# Autodesk Inventor assembly: RotaryBase
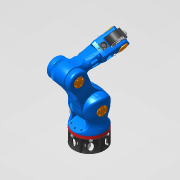
[picture p0: Inventor's stored thumbnail of the model, 180x180]
Saved by Autodesk Inventor 2014 SP2 (Build 180246200, 246)
## iProperties
Created: 2014-12-13
Part Number: RotaryBase
Document SubType Name: Assembly
Designer: 4ndreas
Author: 4ndreas
## Documents named in this file (12)
- C:\Users\4ndreas\Documents\Inventor\RobotARm\RotaryBase.iam
- C:\Users\4ndreas\Documents\Inventor\RobotARm\RotaryBase_B.ipt
- C:\Users\4ndreas\Documents\Inventor\Content Center Files\R2014\de-DE\DIN BEARING(1)\DIN 625 SKF - SKF 608.ipt
- C:\Users\4ndreas\Documents\Inventor\Content Center Files\R2014\de-DE\DIN 931-1\DIN 931-1 - M8 x 60.ipt
- C:\Users\4ndreas\Documents\Inventor\RobotARm\RotaryBase.ipt
- C:\Users\4ndreas\Documents\Inventor\Content Center Files\R2014\de-DE\DIN BEARING(1)\DIN 625 SKF - SKF 625.ipt
- C:\Users\4ndreas\Documents\Inventor\Content Center Files\R2014\de-DE\DIN 931-1\DIN 931-1 - M5 x 25.ipt
- C:\Users\4ndreas\Documents\Inventor\Content Center Files\R2014\de-DE\DIN 985\DIN 985 - M5.ipt
- C:\Users\4ndreas\Documents\Inventor\Content Center Files\R2014\de-DE\DIN 985\DIN 985 - M8.ipt
- C:\Users\4ndreas\Documents\Inventor\RobotARm\Nema17.ipt
- C:\Users\4ndreas\Documents\Inventor\RobotARm\MovingArm.iam
- C:\Users\4ndreas\Documents\Inventor\RobotARm\Stirnzahnrad_C_print.ipt
## Components (27 placed, 11 different names)
1. RotaryBase_B:1 — Fluchtend:1, Passend:1, Passend:2, Passend:3, Passend:4, Passend:5, Passend:6, Passend:8, Passend:9, Passend:13, Passend:16, Passend:17, Passend:18
2. DIN 625 SKF 608:1 — Passend:2, Passend:5
3. DIN 625 SKF 608:2 — Passend:3, Passend:4, Passend:15
4. DIN 931-1 - ersetzt durch DIN EN 24014 M8 x 60:1 — Passend:6, Passend:7, Fluchtend:2, Winkel:1, Passend:14
5. RotaryBase:1 — Passend:7, Tangential:1, Fluchtend:2, Winkel:1, Passend:19, Passend:20, Passend:21
6. DIN 985 - ersetzt durch DIN EN ISO 10511 M8:1 — Passend:14, Passend:15
7. Nema17:1 — Passend:16, Passend:17, Passend:18, Passend:22, Fluchtend:3
8. MovingArm:1 [sub-assembly] — Passend:19, Passend:20, Passend:21
9. Stirnzahnrad_C_print:1 — Passend:22, Fluchtend:3
10. DIN 625 SKF 625:1 — Passend:8, Passend:9, Tangential:1, Passend:10, Passend:11
11. DIN 931-1 - ersetzt durch DIN EN 24014 M5 x 25:1 — Passend:10, Passend:11, Passend:12
12. DIN 985 - ersetzt durch DIN EN ISO 10511 M5:1 — Passend:12, Passend:13
13. DIN 625 SKF 625:2
14. DIN 931-1 - ersetzt durch DIN EN 24014 M5 x 25:2
15. DIN 985 - ersetzt durch DIN EN ISO 10511 M5:2
16. DIN 625 SKF 625:3
17. DIN 931-1 - ersetzt durch DIN EN 24014 M5 x 25:3
18. DIN 985 - ersetzt durch DIN EN ISO 10511 M5:3
19. DIN 625 SKF 625:4
20. DIN 931-1 - ersetzt durch DIN EN 24014 M5 x 25:4
21. DIN 985 - ersetzt durch DIN EN ISO 10511 M5:4
22. DIN 625 SKF 625:5
23. DIN 931-1 - ersetzt durch DIN EN 24014 M5 x 25:5
24. DIN 985 - ersetzt durch DIN EN ISO 10511 M5:5
25. DIN 625 SKF 625:6
26. DIN 931-1 - ersetzt durch DIN EN 24014 M5 x 25:6
27. DIN 985 - ersetzt durch DIN EN ISO 10511 M5:6
## Component patterns: (6 elements, first: DIN 625 SKF 625:1 + DIN 931-1 - ersetzt durch DIN EN 24014 M5 x 25:1 + DIN 985 - ersetzt durch DIN EN ISO 10511 M5:1)
## Relationships (27: Mate 22, Flush 3, Tangent 1, Angle 1)
- Fluchtend:1 [Flush]: RotaryBase_B:1
- Passend:1 [Mate]: RotaryBase_B:1
- Passend:2 [Mate]: RotaryBase_B:1 ↔ DIN 625 SKF 608:1
- Passend:3 [Mate]: RotaryBase_B:1 ↔ DIN 625 SKF 608:2
- Passend:4 [Mate]: RotaryBase_B:1 ↔ DIN 625 SKF 608:2
- Passend:5 [Mate]: RotaryBase_B:1 ↔ DIN 625 SKF 608:1
- Passend:6 [Mate]: RotaryBase_B:1 ↔ DIN 931-1 - ersetzt durch DIN EN 24014 M8 x 60:1
- Passend:7 [Mate]: DIN 931-1 - ersetzt durch DIN EN 24014 M8 x 60:1 ↔ RotaryBase:1
- Passend:8 [Mate]: RotaryBase_B:1 ↔ DIN 625 SKF 625:1
- Passend:9 [Mate]: RotaryBase_B:1 ↔ DIN 625 SKF 625:1
- Tangential:1: RotaryBase:1 ↔ DIN 625 SKF 625:1
- Fluchtend:2 [Flush]: DIN 931-1 - ersetzt durch DIN EN 24014 M8 x 60:1 ↔ RotaryBase:1
- Winkel:1 [Angle] (0 deg): DIN 931-1 - ersetzt durch DIN EN 24014 M8 x 60:1 ↔ RotaryBase:1
- Passend:10 [Mate]: DIN 625 SKF 625:1 ↔ DIN 931-1 - ersetzt durch DIN EN 24014 M5 x 25:1
- Passend:11 [Mate]: DIN 625 SKF 625:1 ↔ DIN 931-1 - ersetzt durch DIN EN 24014 M5 x 25:1
- Passend:12 [Mate]: DIN 931-1 - ersetzt durch DIN EN 24014 M5 x 25:1 ↔ DIN 985 - ersetzt durch DIN EN ISO 10511 M5:1
- Passend:13 [Mate]: RotaryBase_B:1 ↔ DIN 985 - ersetzt durch DIN EN ISO 10511 M5:1
- Passend:14 [Mate]: DIN 931-1 - ersetzt durch DIN EN 24014 M8 x 60:1 ↔ DIN 985 - ersetzt durch DIN EN ISO 10511 M8:1
- Passend:15 [Mate]: DIN 625 SKF 608:2 ↔ DIN 985 - ersetzt durch DIN EN ISO 10511 M8:1
- Passend:16 [Mate]: RotaryBase_B:1 ↔ Nema17:1
- Passend:17 [Mate] (9 mm): RotaryBase_B:1 ↔ Nema17:1
- Passend:18 [Mate]: RotaryBase_B:1 ↔ Nema17:1
- Passend:19 [Mate]: RotaryBase:1 ↔ MovingArm:1
- Passend:20 [Mate]: RotaryBase:1 ↔ MovingArm:1
- Passend:21 [Mate]: RotaryBase:1 ↔ MovingArm:1
- Passend:22 [Mate]: Nema17:1 ↔ Stirnzahnrad_C_print:1
- Fluchtend:3 [Flush]: Nema17:1 ↔ Stirnzahnrad_C_print:1
